# Autodesk Inventor assembly: Vacuum Feed-Through
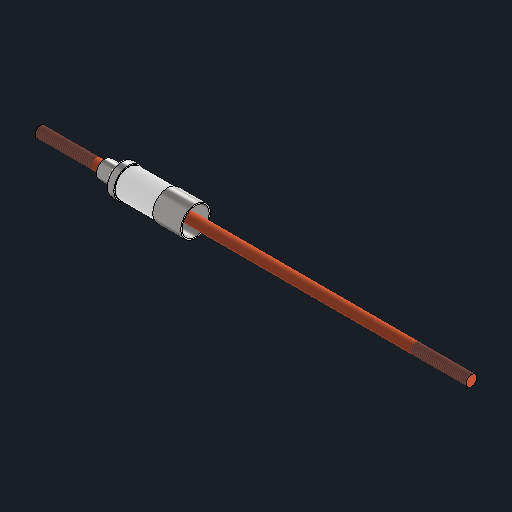
[picture p0: Inventor's stored thumbnail of the model, 512x512]
Saved by Autodesk Inventor 2026 (Build 300175050, 175E)
## iProperties
Created: 2024-05-14
Part Number: Vacuum Feed-Through
Document SubType Name: Assembly
Designer: AK
Mass: 9.25551 g
Surface Area: 46.3476 cm^2
Volume: 5.26495 cm^3
Density: 1.75795 g/cm^3
Author: AK
Title: Vacuum Feed-Through
## Documents named in this file (5)
- C:\Users\queez\Dropbox\Drawings\PIHTI\Plasma Vessel\Cathode-Anode-Flange\copper-feed\HighCurrentFeed.iam
- C:\Users\queez\Dropbox\Drawings\PIHTI\Plasma Vessel\Cathode-Anode-Flange\copper-feed\HighCurrentFeed_Ceramic-insulator.ipt
- C:\Users\queez\Dropbox\Drawings\PIHTI\Plasma Vessel\Cathode-Anode-Flange\copper-feed\HighCurrentFeed_connecting-bushing.ipt
- C:\Users\queez\Dropbox\Drawings\PIHTI\Plasma Vessel\Cathode-Anode-Flange\copper-feed\HighCurrentFeed_welded-plate-top.ipt
- C:\Users\queez\Dropbox\Drawings\PIHTI\Plasma Vessel\Cathode-Anode-Flange\copper-feed\HighCurrentFeedRod.ipt
## Components (4 placed, 4 different names)
1. HighCurrentFeed_Ceramic-insulator:1 — Mate:3, Flush:1, Rigid:1, Rigid:2, Mate:4
2. HighCurrentFeed_connecting-bushing:1 — Rigid:1
3. HighCurrentFeed_welded-plate-top:1 — Rigid:2, Flush:2
4. HighCurrentFeedRod:1 — Mate:4, Flush:2
## Relationships (6: Mate 2, Flush 2, WeldJoint 2)
- Mate:3: HighCurrentFeed_Ceramic-insulator:1
- Flush:1: HighCurrentFeed_Ceramic-insulator:1
- Rigid:1 [WeldJoint] (-2 mm): HighCurrentFeed_Ceramic-insulator:1 ↔ HighCurrentFeed_connecting-bushing:1
- Rigid:2 [WeldJoint]: HighCurrentFeed_Ceramic-insulator:1 ↔ HighCurrentFeed_welded-plate-top:1
- Mate:4: HighCurrentFeed_Ceramic-insulator:1 ↔ HighCurrentFeedRod:1
- Flush:2 (30 mm): HighCurrentFeed_welded-plate-top:1 ↔ HighCurrentFeedRod:1
